# Autodesk Inventor assembly: CoreXY Motor Assembly Right for 4040
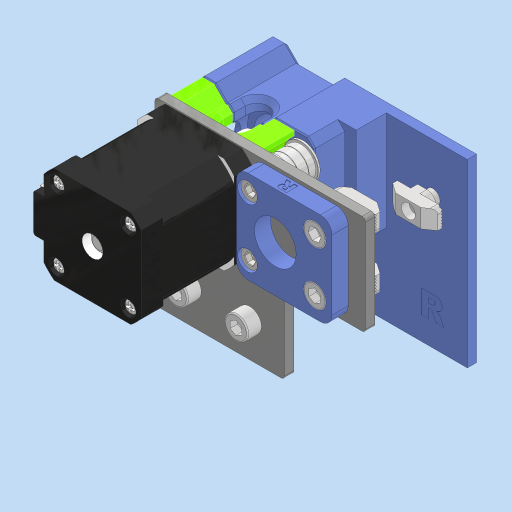
[picture p0: Inventor's stored thumbnail of the model, 512x512]
Saved by Autodesk Inventor 2023.2 (Build 272271000, 271)
## iProperties
Created: 2023-11-27
Part Number: CoreXY Motor Assembly Right for 4040
Document SubType Name: Assembly
Designer: Nils Bade
Author: Nils Bade
## Documents named in this file (16)
- C:\Users\nilsb\Documents\Inventor\Projektarbeit-Bade\RatRig_Bade\CoreXY Motor Assembly Right for 4040.iam
- C:\Users\nilsb\Documents\Inventor\Projektarbeit-Bade\RatRig_modified\xy Motorcage Top Right for 4040.ipt
- C:\Users\nilsb\Documents\Inventor\Projektarbeit-Bade\RatRig_Standards\xy_motor_cage_bottom_right_3.1 v2.ipt
- C:\Users\nilsb\Documents\Inventor\Projektarbeit-Bade\RatRig_modified\Motor Plate Top for 4040.ipt
- C:\Users\nilsb\Documents\Inventor\Projektarbeit-Bade\RatRig_Standards\Nema 17 Stepper Motor - 48mm - 1.8degree_step, 76oz-in v1.ipt
- C:\Users\nilsb\Documents\Inventor\Projektarbeit-Bade\RatRig_Standards\Timing Pulley - 2GT (2mm) - 20 Tooth - For 9mm Belt - 5mm Bo v1.ipt
- C:\Users\nilsb\Documents\Inventor\Projektarbeit-Bade\Schrauben\Cap Head Screw M3x35 v2.ipt
- C:\Users\nilsb\Documents\Inventor\Projektarbeit-Bade\RatRig_modified\T-NUT - DropIn 4040 SERIES - M6.ipt
- C:\Users\nilsb\Documents\Inventor\Projektarbeit-Bade\Schrauben\Cap Head Screw M6x16 - DIN912.ipt
- C:\Users\nilsb\Documents\Inventor\Projektarbeit-Bade\Schrauben\Countersink Screw M6x14 v2.ipt
- C:\Users\nilsb\Documents\Inventor\Projektarbeit-Bade\RatRig_modified\xy Motor Support Right for 4040.ipt
- C:\Users\nilsb\Documents\Inventor\Projektarbeit-Bade\Schrauben\Cap Head Screw M5x40 v2.ipt
- C:\Users\nilsb\Documents\Inventor\Projektarbeit-Bade\RatRig_Standards\Hex Locking Nut - M5 v2.ipt
- C:\Users\nilsb\Documents\Inventor\Projektarbeit-Bade\RatRig_Standards\Mini Precision Shim - 8x5x1mm v2.ipt
- C:\Users\nilsb\Documents\Inventor\Projektarbeit-Bade\RatRig_Standards\Ball Bearing - F695ZZ v1.ipt
- C:\Users\nilsb\Documents\Inventor\Projektarbeit-Bade\RatRig_Standards\Ball Bearing - 695ZZ v1.ipt
## Components (42 placed, 15 different names)
1. xy Motorcage Top Right for 4040:1 — Passend:1, Passend:2, Passend:3, Passend:11, Passend:12, Passend:13, Passend:14, Passend:15, Passend:16, Passend:17, Passend:18, Passend:19, Passend:24, Passend:25, Winkel:3, Winkel:6, Winkel:7, Passend:30, Passend:31, Passend:32, Passend:41, Passend:42, Passend:43, Passend:44, Passend:45, Passend:46, Winkel:10, Winkel:11, Passend:58, Passend:59, Passend:68, Passend:85
2. xy_motor_cage_bottom_right_3.1 v2:1 — Passend:1, Passend:2, Passend:3, Passend:4, Passend:5, Passend:6
3. Motor Plate Top for 4040:1 — Passend:4, Passend:5, Passend:6, Passend:7, Winkel:1, Passend:10, Passend:20, Passend:21, Passend:22, Passend:23, Winkel:4, Winkel:5, Winkel:8, Winkel:9, Passend:26, Passend:27, Passend:28, Passend:29, Passend:33, Passend:34, Passend:35, Passend:36, Passend:39, Passend:40, Passend:47, Passend:48, Passend:49, Passend:66, Passend:73
4. Nema 17 Stepper Motor - 48mm - 1.8degree_step, 76oz-in v1:1 — Passend:7, Winkel:1, Passend:8, Passend:9, Winkel:2, Passend:10
5. Timing Pulley - 2GT (2mm) - 20 Tooth - For 9mm Belt - 5mm Bo v1:1 — Passend:8, Passend:9, Winkel:2
6. Cap Head Screw M3x35 v2:1 — Passend:13, Passend:17
7. Cap Head Screw M3x35 v2:2 — Passend:12, Passend:15
8. Cap Head Screw M3x35 v2:3 — Passend:14, Passend:18
9. Cap Head Screw M3x35 v2:4 — Passend:11, Passend:16
10. T-NUT - DROP IN TYPE FOR 40 SERIES - M6:1 — Passend:20, Winkel:4, Passend:29
11. T-NUT - DROP IN TYPE FOR 40 SERIES - M6:2 — Passend:21, Winkel:5, Passend:28
12. T-NUT - DROP IN TYPE FOR 40 SERIES - M6:3 — Passend:23, Winkel:9, Passend:26
13. T-NUT - DROP IN TYPE FOR 40 SERIES - M6:4 — Passend:22, Winkel:8, Passend:27
14. T-NUT - DROP IN TYPE FOR 40 SERIES - M6:5 — Passend:24, Winkel:6, Passend:31
15. T-NUT - DROP IN TYPE FOR 40 SERIES - M6:6 — Passend:25, Winkel:7, Passend:32
16. T-NUT - DROP IN TYPE FOR 40 SERIES - M6:7 — Passend:19, Winkel:3, Passend:30
17. Cap Head Screw M6x16 - DIN912:1 — Passend:36, Passend:51
18. Cap Head Screw M6x16 - DIN912:2 — Passend:35, Passend:50
19. Cap Head Screw M6x16 - DIN912:3 — Passend:34, Passend:39
20. Cap Head Screw M6x16 - DIN912:4 — Passend:33, Passend:40
21. Countersink Screw M6x14 v2:1 — Passend:43, Passend:45
22. Countersink Screw M6x14 v2:2 — Passend:44, Passend:46
23. Countersink Screw M6x14 v2:3 — Passend:41, Passend:42
24. xy Motor Support Right for 4040:1 — Passend:47, Passend:48, Passend:49, Passend:50, Passend:51, Passend:52, Passend:53, Passend:54, Passend:55
25. Cap Head Screw M5x40 v2:1 — Passend:52, Passend:55, Passend:56, Passend:62, Passend:63, Passend:64, Passend:74, Passend:76, Passend:78, Passend:81, Passend:83, Passend:86
26. Cap Head Screw M5x40 v2:2 — Passend:53, Passend:54, Passend:57, Passend:60, Passend:61, Passend:65, Passend:69, Passend:71
27. Hex Locking Nut - M5 v2:1 — Passend:56, Winkel:10, Passend:59
28. Hex Locking Nut - M5 v2:2 — Passend:57, Winkel:11, Passend:58
29. Mini Precision Shim - 8x5x1mm v2:1 — Passend:60, Passend:66, Passend:67
30. Mini Precision Shim - 8x5x1mm v2:2 — Passend:61, Passend:68
31. Mini Precision Shim - 8x5x1mm v2:3 — Passend:62, Passend:73, Passend:75
32. Mini Precision Shim - 8x5x1mm v2:4 — Passend:63, Passend:80, Passend:82
33. Mini Precision Shim - 8x5x1mm v2:5 — Passend:64, Passend:85
34. Ball Bearing - F695ZZ v1:1 — Passend:86, Passend:87
35. Ball Bearing - F695ZZ v1:2 — Passend:78, Passend:79, Passend:80
36. Ball Bearing - F695ZZ v1:3 — Passend:71, Passend:72
37. Ball Bearing - F695ZZ v1:4 — Passend:81, Passend:82, Passend:84
38. Ball Bearing - F695ZZ v1:5 — Passend:74, Passend:75, Passend:77
39. Ball Bearing - F695ZZ v1:6 — Passend:65, Passend:67, Passend:70
40. Ball Bearing - 695ZZ v1:1 — Passend:69, Passend:70, Passend:72
41. Ball Bearing - 695ZZ v1:2 — Passend:76, Passend:77, Passend:79
42. Ball Bearing - 695ZZ v1:3 — Passend:83, Passend:84, Passend:87
## Relationships (96: Mate 85, Angle 11)
- Passend:1 [Mate]: xy Motorcage Top Right for 4040:1 ↔ xy_motor_cage_bottom_right_3.1 v2:1
- Passend:2 [Mate]: xy Motorcage Top Right for 4040:1 ↔ xy_motor_cage_bottom_right_3.1 v2:1
- Passend:3 [Mate]: xy Motorcage Top Right for 4040:1 ↔ xy_motor_cage_bottom_right_3.1 v2:1
- Passend:4 [Mate]: xy_motor_cage_bottom_right_3.1 v2:1 ↔ Motor Plate Top for 4040:1
- Passend:5 [Mate]: xy_motor_cage_bottom_right_3.1 v2:1 ↔ Motor Plate Top for 4040:1
- Passend:6 [Mate]: xy_motor_cage_bottom_right_3.1 v2:1 ↔ Motor Plate Top for 4040:1
- Passend:7 [Mate]: Motor Plate Top for 4040:1 ↔ Nema 17 Stepper Motor - 48mm - 1.8degree_step, 76oz-in v1:1
- Winkel:1 [Angle] (0 deg): Motor Plate Top for 4040:1 ↔ Nema 17 Stepper Motor - 48mm - 1.8degree_step, 76oz-in v1:1
- Passend:8 [Mate]: Nema 17 Stepper Motor - 48mm - 1.8degree_step, 76oz-in v1:1 ↔ Timing Pulley - 2GT (2mm) - 20 Tooth - For 9mm Belt - 5mm Bo v1:1
- Passend:9 [Mate] (1 mm): Nema 17 Stepper Motor - 48mm - 1.8degree_step, 76oz-in v1:1 ↔ Timing Pulley - 2GT (2mm) - 20 Tooth - For 9mm Belt - 5mm Bo v1:1
- Winkel:2 [Angle] (0 deg): Nema 17 Stepper Motor - 48mm - 1.8degree_step, 76oz-in v1:1 ↔ Timing Pulley - 2GT (2mm) - 20 Tooth - For 9mm Belt - 5mm Bo v1:1
- Passend:10 [Mate]: Motor Plate Top for 4040:1 ↔ Nema 17 Stepper Motor - 48mm - 1.8degree_step, 76oz-in v1:1
- Passend:11 [Mate]: xy Motorcage Top Right for 4040:1 ↔ Cap Head Screw M3x35 v2:4
- Passend:12 [Mate]: xy Motorcage Top Right for 4040:1 ↔ Cap Head Screw M3x35 v2:2
- Passend:13 [Mate]: xy Motorcage Top Right for 4040:1 ↔ Cap Head Screw M3x35 v2:1
- Passend:14 [Mate]: xy Motorcage Top Right for 4040:1 ↔ Cap Head Screw M3x35 v2:3
- Passend:15 [Mate]: xy Motorcage Top Right for 4040:1 ↔ Cap Head Screw M3x35 v2:2
- Passend:16 [Mate]: xy Motorcage Top Right for 4040:1 ↔ Cap Head Screw M3x35 v2:4
- Passend:17 [Mate]: xy Motorcage Top Right for 4040:1 ↔ Cap Head Screw M3x35 v2:1
- Passend:18 [Mate]: xy Motorcage Top Right for 4040:1 ↔ Cap Head Screw M3x35 v2:3
- Passend:19 [Mate]: xy Motorcage Top Right for 4040:1 ↔ T-NUT - DROP IN TYPE FOR 40 SERIES - M6:7
- Passend:20 [Mate]: Motor Plate Top for 4040:1 ↔ T-NUT - DROP IN TYPE FOR 40 SERIES - M6:1
- Passend:21 [Mate]: Motor Plate Top for 4040:1 ↔ T-NUT - DROP IN TYPE FOR 40 SERIES - M6:2
- Passend:22 [Mate]: Motor Plate Top for 4040:1 ↔ T-NUT - DROP IN TYPE FOR 40 SERIES - M6:4
- Passend:23 [Mate]: Motor Plate Top for 4040:1 ↔ T-NUT - DROP IN TYPE FOR 40 SERIES - M6:3
- Passend:24 [Mate]: xy Motorcage Top Right for 4040:1 ↔ T-NUT - DROP IN TYPE FOR 40 SERIES - M6:5
- Passend:25 [Mate]: xy Motorcage Top Right for 4040:1 ↔ T-NUT - DROP IN TYPE FOR 40 SERIES - M6:6
- Winkel:3 [Angle] (0 deg): xy Motorcage Top Right for 4040:1 ↔ T-NUT - DROP IN TYPE FOR 40 SERIES - M6:7
- Winkel:4 [Angle] (0 deg): Motor Plate Top for 4040:1 ↔ T-NUT - DROP IN TYPE FOR 40 SERIES - M6:1
- Winkel:5 [Angle] (0 deg): Motor Plate Top for 4040:1 ↔ T-NUT - DROP IN TYPE FOR 40 SERIES - M6:2
- Winkel:6 [Angle] (0 deg): xy Motorcage Top Right for 4040:1 ↔ T-NUT - DROP IN TYPE FOR 40 SERIES - M6:5
- Winkel:7 [Angle] (0 deg): xy Motorcage Top Right for 4040:1 ↔ T-NUT - DROP IN TYPE FOR 40 SERIES - M6:6
- Winkel:8 [Angle] (0 deg): Motor Plate Top for 4040:1 ↔ T-NUT - DROP IN TYPE FOR 40 SERIES - M6:4
- Winkel:9 [Angle] (0 deg): Motor Plate Top for 4040:1 ↔ T-NUT - DROP IN TYPE FOR 40 SERIES - M6:3
- Passend:26 [Mate] (5.5 mm): Motor Plate Top for 4040:1 ↔ T-NUT - DROP IN TYPE FOR 40 SERIES - M6:3
- Passend:27 [Mate] (5.5 mm): Motor Plate Top for 4040:1 ↔ T-NUT - DROP IN TYPE FOR 40 SERIES - M6:4
- Passend:28 [Mate] (5.5 mm): Motor Plate Top for 4040:1 ↔ T-NUT - DROP IN TYPE FOR 40 SERIES - M6:2
- Passend:29 [Mate] (5.5 mm): Motor Plate Top for 4040:1 ↔ T-NUT - DROP IN TYPE FOR 40 SERIES - M6:1
- Passend:30 [Mate] (5.5 mm): xy Motorcage Top Right for 4040:1 ↔ T-NUT - DROP IN TYPE FOR 40 SERIES - M6:7
- Passend:31 [Mate] (5.5 mm): xy Motorcage Top Right for 4040:1 ↔ T-NUT - DROP IN TYPE FOR 40 SERIES - M6:5
- Passend:32 [Mate] (5.5 mm): xy Motorcage Top Right for 4040:1 ↔ T-NUT - DROP IN TYPE FOR 40 SERIES - M6:6
- Passend:33 [Mate]: Motor Plate Top for 4040:1 ↔ Cap Head Screw M6x16 - DIN912:4
- Passend:34 [Mate]: Motor Plate Top for 4040:1 ↔ Cap Head Screw M6x16 - DIN912:3
- Passend:35 [Mate]: Motor Plate Top for 4040:1 ↔ Cap Head Screw M6x16 - DIN912:2
- Passend:36 [Mate]: Motor Plate Top for 4040:1 ↔ Cap Head Screw M6x16 - DIN912:1
- Passend:39 [Mate]: Motor Plate Top for 4040:1 ↔ Cap Head Screw M6x16 - DIN912:3
- Passend:40 [Mate]: Motor Plate Top for 4040:1 ↔ Cap Head Screw M6x16 - DIN912:4
- Passend:41 [Mate]: xy Motorcage Top Right for 4040:1 ↔ Countersink Screw M6x14 v2:3
- Passend:42 [Mate]: xy Motorcage Top Right for 4040:1 ↔ Countersink Screw M6x14 v2:3
- Passend:43 [Mate]: xy Motorcage Top Right for 4040:1 ↔ Countersink Screw M6x14 v2:1
- Passend:44 [Mate]: xy Motorcage Top Right for 4040:1 ↔ Countersink Screw M6x14 v2:2
- Passend:45 [Mate]: xy Motorcage Top Right for 4040:1 ↔ Countersink Screw M6x14 v2:1
- Passend:46 [Mate]: xy Motorcage Top Right for 4040:1 ↔ Countersink Screw M6x14 v2:2
- Passend:47 [Mate]: Motor Plate Top for 4040:1 ↔ xy Motor Support Right for 4040:1
- Passend:48 [Mate]: Motor Plate Top for 4040:1 ↔ xy Motor Support Right for 4040:1
- Passend:49 [Mate]: Motor Plate Top for 4040:1 ↔ xy Motor Support Right for 4040:1
- Passend:50 [Mate]: Cap Head Screw M6x16 - DIN912:2 ↔ xy Motor Support Right for 4040:1
- Passend:51 [Mate]: Cap Head Screw M6x16 - DIN912:1 ↔ xy Motor Support Right for 4040:1
- Passend:52 [Mate]: xy Motor Support Right for 4040:1 ↔ Cap Head Screw M5x40 v2:1
- Passend:53 [Mate]: xy Motor Support Right for 4040:1 ↔ Cap Head Screw M5x40 v2:2
- Passend:54 [Mate]: xy Motor Support Right for 4040:1 ↔ Cap Head Screw M5x40 v2:2
- Passend:55 [Mate]: xy Motor Support Right for 4040:1 ↔ Cap Head Screw M5x40 v2:1
- Passend:56 [Mate]: Cap Head Screw M5x40 v2:1 ↔ Hex Locking Nut - M5 v2:1
- Passend:57 [Mate]: Cap Head Screw M5x40 v2:2 ↔ Hex Locking Nut - M5 v2:2
- Winkel:10 [Angle] (0 deg): xy Motorcage Top Right for 4040:1 ↔ Hex Locking Nut - M5 v2:1
- Winkel:11 [Angle] (0 deg): xy Motorcage Top Right for 4040:1 ↔ Hex Locking Nut - M5 v2:2
- Passend:58 [Mate]: xy Motorcage Top Right for 4040:1 ↔ Hex Locking Nut - M5 v2:2
- Passend:59 [Mate]: xy Motorcage Top Right for 4040:1 ↔ Hex Locking Nut - M5 v2:1
- Passend:60 [Mate]: Cap Head Screw M5x40 v2:2 ↔ Mini Precision Shim - 8x5x1mm v2:1
- Passend:61 [Mate]: Cap Head Screw M5x40 v2:2 ↔ Mini Precision Shim - 8x5x1mm v2:2
- Passend:62 [Mate]: Cap Head Screw M5x40 v2:1 ↔ Mini Precision Shim - 8x5x1mm v2:3
- Passend:63 [Mate]: Cap Head Screw M5x40 v2:1 ↔ Mini Precision Shim - 8x5x1mm v2:4
- Passend:64 [Mate]: Cap Head Screw M5x40 v2:1 ↔ Mini Precision Shim - 8x5x1mm v2:5
- Passend:65 [Mate]: Cap Head Screw M5x40 v2:2 ↔ Ball Bearing - F695ZZ v1:6
- Passend:66 [Mate]: Motor Plate Top for 4040:1 ↔ Mini Precision Shim - 8x5x1mm v2:1
- Passend:67 [Mate]: Mini Precision Shim - 8x5x1mm v2:1 ↔ Ball Bearing - F695ZZ v1:6
- Passend:68 [Mate]: xy Motorcage Top Right for 4040:1 ↔ Mini Precision Shim - 8x5x1mm v2:2
- Passend:69 [Mate]: Cap Head Screw M5x40 v2:2 ↔ Ball Bearing - 695ZZ v1:1
- Passend:70 [Mate]: Ball Bearing - F695ZZ v1:6 ↔ Ball Bearing - 695ZZ v1:1
- Passend:71 [Mate]: Cap Head Screw M5x40 v2:2 ↔ Ball Bearing - F695ZZ v1:3
- Passend:72 [Mate]: Ball Bearing - F695ZZ v1:3 ↔ Ball Bearing - 695ZZ v1:1
- Passend:73 [Mate]: Motor Plate Top for 4040:1 ↔ Mini Precision Shim - 8x5x1mm v2:3
- Passend:74 [Mate]: Cap Head Screw M5x40 v2:1 ↔ Ball Bearing - F695ZZ v1:5
- Passend:75 [Mate]: Mini Precision Shim - 8x5x1mm v2:3 ↔ Ball Bearing - F695ZZ v1:5
- Passend:76 [Mate]: Cap Head Screw M5x40 v2:1 ↔ Ball Bearing - 695ZZ v1:2
- Passend:77 [Mate]: Ball Bearing - F695ZZ v1:5 ↔ Ball Bearing - 695ZZ v1:2
- Passend:78 [Mate]: Cap Head Screw M5x40 v2:1 ↔ Ball Bearing - F695ZZ v1:2
- Passend:79 [Mate]: Ball Bearing - F695ZZ v1:2 ↔ Ball Bearing - 695ZZ v1:2
- Passend:80 [Mate]: Mini Precision Shim - 8x5x1mm v2:4 ↔ Ball Bearing - F695ZZ v1:2
- Passend:81 [Mate]: Cap Head Screw M5x40 v2:1 ↔ Ball Bearing - F695ZZ v1:4
- Passend:82 [Mate]: Mini Precision Shim - 8x5x1mm v2:4 ↔ Ball Bearing - F695ZZ v1:4
- Passend:83 [Mate]: Cap Head Screw M5x40 v2:1 ↔ Ball Bearing - 695ZZ v1:3
- Passend:84 [Mate]: Ball Bearing - F695ZZ v1:4 ↔ Ball Bearing - 695ZZ v1:3
- Passend:85 [Mate]: xy Motorcage Top Right for 4040:1 ↔ Mini Precision Shim - 8x5x1mm v2:5
- Passend:86 [Mate]: Cap Head Screw M5x40 v2:1 ↔ Ball Bearing - F695ZZ v1:1
- Passend:87 [Mate]: Ball Bearing - F695ZZ v1:1 ↔ Ball Bearing - 695ZZ v1:3
